# Autodesk Inventor assembly: pulleyassebly
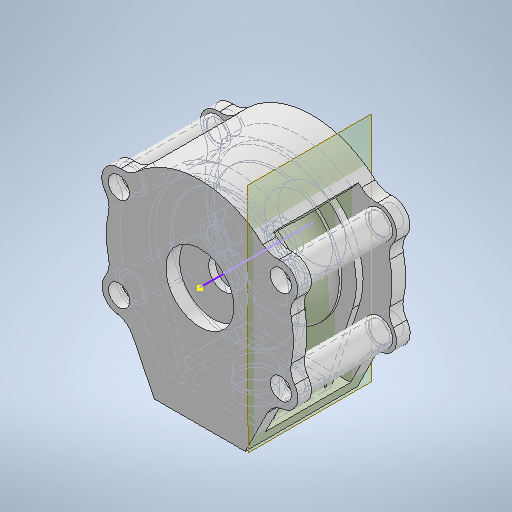
[picture p0: Inventor's stored thumbnail of the model, 512x512]
Saved by Autodesk Inventor 2025.2 (Build 292293000, 293)
## iProperties
Created: 2025-01-13
Part Number: pulleyassebly
Document SubType Name: Assembly
Designer: email
Author: email
## Documents named in this file (5)
- C:\Users\email\Desktop\Projects\Capstone\4TB6\CAD_Model\thigh_mount\pulleyassebly.iam
- C:\Users\email\Desktop\Projects\Capstone\4TB6\CAD_Model\pidtest\pulley.ipt
- C:\Users\email\Desktop\Projects\Capstone\4TB6\CAD_Model\pidtest\pulleybearing.ipt
- C:\Users\email\Desktop\Projects\Capstone\4TB6\CAD_Model\thigh_mount\pulleyblocker.ipt
- C:\Users\email\Desktop\Projects\Capstone\4TB6\CAD_Model\thigh_mount\pulleyspacer.ipt
## Components (7 placed, 4 different names)
1. pulley:1 — Mate:1, Mate:2, Mate:3, Mate:4
2. pulleybearing:1 — Mate:1, Mate:2
3. pulleyblocker:1 — Mate:3, Mate:4, Mate:5, Mate:6, Mate:7, Mate:8, Mate:9, Mate:10, Mate:11, Mate:12
4. pulleyspacer:1 — Mate:6, Mate:11
5. pulleyspacer:2 — Mate:8, Mate:12
6. pulleyspacer:3 — Mate:5, Mate:10
7. pulleyspacer:4 — Mate:7, Mate:9
## Relationships (12: Mate 12)
- Mate:1: pulley:1 ↔ pulleybearing:1
- Mate:2 (1 mm): pulley:1 ↔ pulleybearing:1
- Mate:3: pulley:1 ↔ pulleyblocker:1
- Mate:4 (3 mm): pulley:1 ↔ pulleyblocker:1
- Mate:5: pulleyblocker:1 ↔ pulleyspacer:3
- Mate:6: pulleyblocker:1 ↔ pulleyspacer:1
- Mate:7: pulleyblocker:1 ↔ pulleyspacer:4
- Mate:8: pulleyblocker:1 ↔ pulleyspacer:2
- Mate:9: pulleyblocker:1 ↔ pulleyspacer:4
- Mate:10: pulleyblocker:1 ↔ pulleyspacer:3
- Mate:11: pulleyblocker:1 ↔ pulleyspacer:1
- Mate:12: pulleyblocker:1 ↔ pulleyspacer:2
